# Autodesk Inventor assembly: robotetz
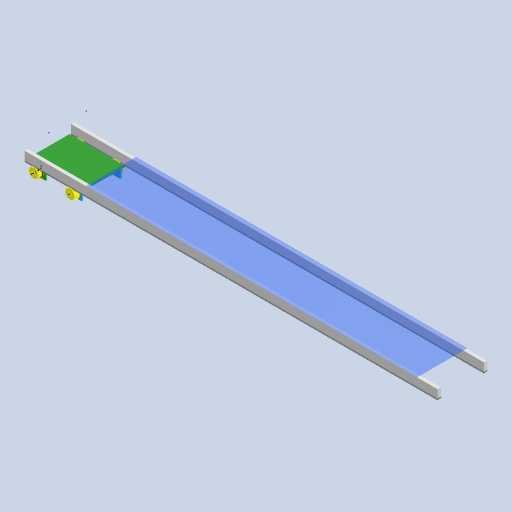
[picture p0: Inventor's stored thumbnail of the model, 512x512]
Saved by Autodesk Inventor 2024.2 (Build 282272000, 272)
## iProperties
Created: 2025-11-16
Part Number: robotetz
Document SubType Name: Assembly
Designer: katya_notebook
Author: katya_notebook
## Documents named in this file (23)
- C:\Users\91125\OneDrive\Рабочий стол\alletz\3д модель\etz\robotetz.iam
- C:\Users\91125\OneDrive\Рабочий стол\alletz\3д модель\полигон\полигон етз.iam
- C:\Users\91125\OneDrive\Рабочий стол\alletz\3д модель\Шестерня.ipt
- C:\Users\91125\OneDrive\Рабочий стол\alletz\3д модель\муфта.ipt
- C:\Users\91125\OneDrive\Рабочий стол\alletz\3д модель\Шестерня_MIR.ipt
- C:\Users\91125\OneDrive\Рабочий стол\alletz\3д модель\муфта_MIR.ipt
- C:\Users\91125\OneDrive\Рабочий стол\alletz\3д модель\мотор левая.iam
- C:\Users\91125\OneDrive\Рабочий стол\alletz\3д модель\мотор левая_MIR.iam
- C:\Users\91125\OneDrive\Рабочий стол\alletz\3д модель\нижняя пластина.ipt
- C:\Users\91125\OneDrive\Рабочий стол\alletz\3д модель\верхняя пластина.ipt
- C:\Users\91125\OneDrive\Рабочий стол\alletz\3д модель\крепление свободной шестерни.ipt
- C:\Users\91125\OneDrive\Рабочий стол\alletz\3д модель\Шестерня_MIR1.ipt
- C:\Users\91125\OneDrive\Рабочий стол\alletz\3д модель\Шестерня_MIR_MIR.ipt
- C:\Users\91125\OneDrive\Рабочий стол\alletz\3д модель\вал.ipt
- C:\Users\91125\OneDrive\Рабочий стол\alletz\3д модель\вал_MIR.ipt
- C:\Users\91125\OneDrive\Рабочий стол\alletz\3д модель\муфта_MIR1.ipt
- C:\Users\91125\OneDrive\Рабочий стол\alletz\3д модель\муфта_MIR_MIR.ipt
- C:\Users\91125\OneDrive\Рабочий стол\alletz\3д модель\цили.ipt
- C:\Users\91125\OneDrive\Рабочий стол\alletz\3д модель\подшипник.ipt
- C:\Users\91125\OneDrive\Рабочий стол\alletz\3д модель\верх штуки для подшипников.ipt
- C:\Users\91125\OneDrive\Рабочий стол\alletz\3д модель\крепление свободной шестерни_MIR.ipt
- C:\Users\91125\OneDrive\Рабочий стол\alletz\3д модель\цили_MIR.ipt
- C:\Users\91125\OneDrive\Рабочий стол\alletz\3д модель\верх штуки для подшипников_MIR.ipt
## Components (22 placed, 22 different names)
1. полигон етз:1 [sub-assembly] — Заподлицо:1, Совмещение:1, Заподлицо:3, Заподлицо:8
2. Шестерня:1 — Заподлицо:1, Совмещение:1, С поворотом:1
3. муфта:1 — С поворотом:1, С поворотом:3
4. Шестерня_MIR:1 — С поворотом:2
5. муфта_MIR:1 — С поворотом:2
6. мотор левая:1 [sub-assembly] — С поворотом:3, Заподлицо:3, Заподлицо:9, Заподлицо:11
7. мотор левая_MIR:1 [sub-assembly] — Заподлицо:10
8. нижняя пластина:1 — Заподлицо:9, Заподлицо:12
9. верхняя пластина:1 — Заподлицо:10, Заподлицо:11, Заподлицо:13
10. Шестерня_MIR1:1
11. Шестерня_MIR_MIR:1 — Заподлицо:14
12. вал:1 — Заподлицо:14
13. вал_MIR:1
14. муфта_MIR1:1
15. муфта_MIR_MIR:1
16. подшипник:1 — Цилиндрический:1
17. крепление свободной шестерни:1 — Заподлицо:12, Заподлицо:16, Заподлицо:18
18. цили:1 — Заподлицо:16, Цилиндрический:1, Заподлицо:17
19. верх штуки для подшипников:1 — Заподлицо:17, Заподлицо:18
20. крепление свободной шестерни_MIR:1 — Совмещение:2, Совмещение:3
21. цили_MIR:1 — Совмещение:2, Совмещение:4
22. верх штуки для подшипников_MIR:1 — Совмещение:3, Совмещение:4
## Relationships (24: Flush 15, Mate 4, RevoluteJoint 3, WeldJoint 1, CylindricalJoint 1)
- Заподлицо:1 [Flush]: полигон етз:1 ↔ Шестерня:1
- Совмещение:1 [Mate] (28 mm): полигон етз:1 ↔ Шестерня:1
- С поворотом:1 [RevoluteJoint]: Шестерня:1 ↔ муфта:1
- С поворотом:2 [RevoluteJoint]: Шестерня_MIR:1 ↔ муфта_MIR:1
- С поворотом:3 [RevoluteJoint]: муфта:1 ↔ мотор левая:1
- [WeldJoint]: муфта_MIR:1 ↔ мотор левая_MIR:1
- [Flush]: мотор левая:1 ↔ мотор левая_MIR:1
- Заподлицо:3 [Flush]: полигон етз:1 ↔ мотор левая:1
- [Flush]: мотор левая:1 ↔ мотор левая_MIR:1
- [Flush]: мотор левая:1 ↔ мотор левая_MIR:1
- Заподлицо:8 [Flush] (105 mm): полигон етз:1
- Заподлицо:9 [Flush]: мотор левая:1 ↔ нижняя пластина:1
- Заподлицо:10 [Flush]: мотор левая_MIR:1 ↔ верхняя пластина:1
- Заподлицо:11 [Flush]: мотор левая:1 ↔ верхняя пластина:1
- Заподлицо:12 [Flush]: нижняя пластина:1 ↔ крепление свободной шестерни:1
- Заподлицо:13 [Flush] (-135 mm): верхняя пластина:1
- Заподлицо:14 [Flush]: Шестерня_MIR_MIR:1 ↔ вал:1
- Заподлицо:16 [Flush] (-30 mm): крепление свободной шестерни:1 ↔ цили:1
- Цилиндрический:1 [CylindricalJoint]: подшипник:1 ↔ цили:1
- Заподлицо:17 [Flush]: цили:1 ↔ верх штуки для подшипников:1
- Заподлицо:18 [Flush]: крепление свободной шестерни:1 ↔ верх штуки для подшипников:1
- Совмещение:2 [Mate] (-30 mm): крепление свободной шестерни_MIR:1 ↔ цили_MIR:1
- Совмещение:3 [Mate]: крепление свободной шестерни_MIR:1 ↔ верх штуки для подшипников_MIR:1
- Совмещение:4 [Mate]: цили_MIR:1 ↔ верх штуки для подшипников_MIR:1
